# Autodesk Inventor assembly: top_2
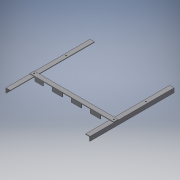
[picture p0: Inventor's stored thumbnail of the model, 180x180]
Saved by Autodesk Inventor 2017 (Build 210142000, 142)
## iProperties
Created: 2018-10-22
Part Number: top_2
Document SubType Name: Assembly
Designer: ddeboer
Author: ddeboer
## Documents named in this file (3)
- C:\Users\ddeboer\Desktop\snap_holder\top_2.iam
- C:\Users\ddeboer\Desktop\snap_holder\angle_L103.ipt
- C:\Users\ddeboer\Desktop\snap_holder\angle_L101.ipt
## Components (3 placed, 2 different names)
1. angle_L103:1 — Insert:1, Flush:1, Insert:2, Flush:2
2. angle_L101:1 — Insert:1, Flush:1
3. angle_L101:2 — Insert:2, Flush:2
## Relationships (4: Insert 2, Flush 2)
- Insert:1: angle_L103:1 ↔ angle_L101:1
- Flush:1: angle_L103:1 ↔ angle_L101:1
- Insert:2: angle_L103:1 ↔ angle_L101:2
- Flush:2: angle_L103:1 ↔ angle_L101:2
